# Autodesk Inventor assembly: oled assy
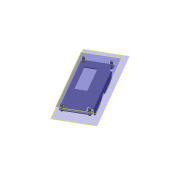
[picture p0: Inventor's stored thumbnail of the model, 180x180]
Saved by Autodesk Inventor 2016 (Build 200138000, 138)
## iProperties
Created: 2016-08-18
Part Number: oled assy
Document SubType Name: Assembly
Designer: admin
Author: admin
## Documents named in this file (4)
- C:\Users\Juny\Desktop\Ateam\1612 3D 도면\oled assy\oled assy.iam
- C:\Users\Juny\Desktop\Ateam\1612 3D 도면\oled assy\m3 6 socket_screw.ipt
- C:\Users\Juny\Desktop\Ateam\1612 3D 도면\oled assy\m3 10 pcb_support.ipt
- C:\Users\Juny\Desktop\Ateam\1612 3D 도면\oled assy\oled_Brackets.ipt
## Components (9 placed, 3 different names)
1. m3 6 socket_screw:1 — Rotational:7
2. m3 10 pcb_support:1 — Rotational:6
3. oled_Brackets:1 — Rotational:5, Rotational:6, Rotational:7, Rotational:8, Rotational:9, Rotational:10
4. m3 10 pcb_support:2
5. m3 10 pcb_support:3
6. m3 10 pcb_support:4 — Rotational:5
7. m3 6 socket_screw:2 — Rotational:8
8. m3 6 socket_screw:3 — Rotational:9
9. m3 6 socket_screw:4 — Rotational:10
## Relationships (6: RevoluteJoint 6)
- Rotational:5 [RevoluteJoint]: oled_Brackets:1 ↔ m3 10 pcb_support:4
- Rotational:6 [RevoluteJoint]: m3 10 pcb_support:1 ↔ oled_Brackets:1
- Rotational:7 [RevoluteJoint]: m3 6 socket_screw:1 ↔ oled_Brackets:1
- Rotational:8 [RevoluteJoint]: oled_Brackets:1 ↔ m3 6 socket_screw:2
- Rotational:9 [RevoluteJoint]: oled_Brackets:1 ↔ m3 6 socket_screw:3
- Rotational:10 [RevoluteJoint]: oled_Brackets:1 ↔ m3 6 socket_screw:4
